# Autodesk Inventor assembly: NavCom
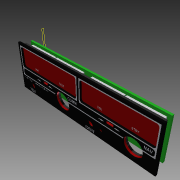
[picture p0: Inventor's stored thumbnail of the model, 180x180]
Saved by Autodesk Inventor 2014 (Build 180170000, 170)
## iProperties
Created: 2017-02-12
Part Number: NavCom
Document SubType Name: Assembly
Designer: N
Author: N
## Documents named in this file (5)
- D:\Projekty\RadioStack_v2\Vykresy\Inventor\NavCom.iam
- D:\Projekty\RadioStack_v2\Vykresy\Inventor\NavCom_mask.ipt
- D:\Projekty\RadioStack_v2\Vykresy\Inventor\NavCom_plexi.ipt
- D:\Projekty\RadioStack_v2\Vykresy\Inventor\NavCom_panel.ipt
- D:\Projekty\RadioStack_v2\Vykresy\Inventor\NavCom_PCB.ipt
## Components (4 placed, 4 different names)
1. NavCom_mask:1 — Proti sobě:3, Stejný směr:3, Stejný směr:4
2. NavCom_plexi:1 — Proti sobě:2, Stejný směr:1, Stejný směr:2, Proti sobě:3, Stejný směr:3, Stejný směr:4
3. NavCom_panel:1
4. NavCom_PCB:1 — Proti sobě:2, Stejný směr:1, Stejný směr:2
## Relationships (6: Flush 4, Mate 2)
- Proti sobě:2 [Mate]: NavCom_plexi:1 ↔ NavCom_PCB:1
- Stejný směr:1 [Flush]: NavCom_plexi:1 ↔ NavCom_PCB:1
- Stejný směr:2 [Flush]: NavCom_plexi:1 ↔ NavCom_PCB:1
- Proti sobě:3 [Mate]: NavCom_mask:1 ↔ NavCom_plexi:1
- Stejný směr:3 [Flush]: NavCom_mask:1 ↔ NavCom_plexi:1
- Stejný směr:4 [Flush]: NavCom_mask:1 ↔ NavCom_plexi:1
